# Autodesk Inventor assembly: 2016-02-08-RobotV15
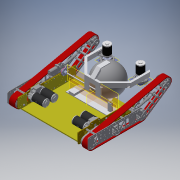
[picture p0: Inventor's stored thumbnail of the model, 180x180]
Saved by Autodesk Inventor 2016 SP1 (Build 200210100, 210)
## iProperties
Created: 2016-02-10
Part Number: 2016-02-08-RobotV15
Document SubType Name: Assembly
Designer: steele
Author: steele
## Documents named in this file (5)
- C:\snobotics\CAD-Development\robSteele\SnoBotics2016\2016-02-08-RhinoTrackWithSheetBase\2016-02-08-RobotV15.iam
- C:\snobotics\CAD-Development\robSteele\SnoBotics2016\RhinoTrackDriveModule\am-3322+RhinoTrackDriveModule.iam
- C:\snobotics\CAD-Development\robSteele\SnoBotics2016\RhinoBottomFloorOptions\SheetBottomFloorV01.ipt
- C:\snobotics\CAD-Development\robSteele\SnoBotics2016\RhinoTrackDriveModule\am-3322+RhinoTrackDriveModule_MIR13.iam
- C:\snobotics\CAD-Development\robSteele\SnoBotics2016\2016-05-05-ShooterPrototype\ShooterAssemblyV05.iam
## Components (4 placed, 4 different names)
1. am-3322+RhinoTrackDriveModule:1 [sub-assembly] — Mate:1, Flush:1, Flush:2
2. SheetBottomFloorV01:1 — Mate:1, Flush:1, Flush:2, Mate:2, Mate:3, Flush:3
3. am-3322+RhinoTrackDriveModule_MIR13:1 [sub-assembly]
4. ShooterAssemblyV05:1 [sub-assembly] — Mate:2, Mate:3, Flush:3
## Relationships (6: Mate 3, Flush 3)
- Mate:1: am-3322+RhinoTrackDriveModule:1 ↔ SheetBottomFloorV01:1
- Flush:1: am-3322+RhinoTrackDriveModule:1 ↔ SheetBottomFloorV01:1
- Flush:2 (4.7625 mm): am-3322+RhinoTrackDriveModule:1 ↔ SheetBottomFloorV01:1
- Mate:2: SheetBottomFloorV01:1 ↔ ShooterAssemblyV05:1
- Mate:3: SheetBottomFloorV01:1 ↔ ShooterAssemblyV05:1
- Flush:3 (-63.5 mm): SheetBottomFloorV01:1 ↔ ShooterAssemblyV05:1
